# Autodesk Inventor assembly: TBone Cart
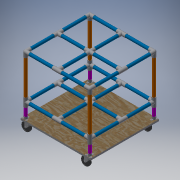
[picture p0: Inventor's stored thumbnail of the model, 180x180]
Saved by Autodesk Inventor 2018.2 (Build 222227000, 227)
## iProperties
Created: 2018-02-01
Part Number: TBone Cart
Document SubType Name: Assembly
Designer: owner
Author: owner
## Documents named in this file (11)
- Z:\The Pickle - 4 - Copy\Final Carts\T-Bone Cart\T-Bone Cart.iam
- Z:\The Pickle - 4 - Copy\Final Carts\Stuff Used By All Carts\PVC Fittings (Formufit)\4-way Tee 1 Inch.ipt
- Z:\The Pickle - 4 - Copy\Final Carts\Stuff Used By All Carts\PVC Fittings (Formufit)\Tee 1 Inch.ipt
- Z:\The Pickle - 4 - Copy\Final Carts\Stuff Used By All Carts\PVC Fittings (Formufit)\Cross 1 Inch.ipt
- Z:\The Pickle - 4 - Copy\Final Carts\Stuff Used By All Carts\PVC Fittings (Formufit)\Wood Mount 1 Inch.ipt
- Z:\The Pickle\Final Carts\T-Bone Cart\Pipe 1.ipt
- Z:\The Pickle\Final Carts\T-Bone Cart\Pipe 2.ipt
- Z:\The Pickle\Final Carts\T-Bone Cart\Pipe 3.ipt
- Z:\The Pickle - 4 - Copy\Final Carts\Stuff Used By All Carts\WHEELS.ipt
- Z:\The Pickle - 4 - Copy\Final Carts\Stuff Used By All Carts\PVC Fittings (Formufit)\3-way 90 1 Inch.ipt
- Z:\The Pickle - 4 - Copy\Final Carts\T-Bone Cart\T-Bone Plywood Base.ipt
## Components (59 placed, 10 different names)
1. T-Bone Plywood Base:1 — Mate:1, Tangent:1, Tangent:2, Flush:8, Flush:9, Flush:10, Flush:11, Mate:2, Tangent:3, Tangent:4, Tangent:5, Tangent:6, Tangent:7, Angle:1
2. 4-way Tee 1 Inch:1 — Insert:11, Insert:12, Insert:29, Insert:33
3. 4-way Tee 1 Inch:2 — Insert:7, Insert:8, Insert:28, Insert:32
4. 4-way Tee 1 Inch:3 — Insert:2, Insert:3, Insert:4, Insert:19
5. 4-way Tee 1 Inch:4 — Insert:15, Insert:16, Insert:30, Insert:31
6. Tee 1 Inch:1 — Insert:46, Insert:53
7. Tee 1 Inch:2 — Insert:13, Insert:14, Insert:21
8. Tee 1 Inch:3 — Insert:17, Insert:18, Insert:22
9. Tee 1 Inch:4 — Insert:47, Insert:52
10. Tee 1 Inch:5 — Insert:5, Insert:6, Insert:20
11. Tee 1 Inch:6 — Insert:49, Insert:51
12. Tee 1 Inch:7 — Insert:48, Insert:50
13. Tee 1 Inch:8 — Insert:9, Insert:10, Insert:23
14. Cross 1 Inch:1 — Insert:54, Insert:59
15. Cross 1 Inch:2 — Insert:24
16. Wood Mount 1 Inch:1 — Insert:25, Tangent:6
17. Wood Mount 1 Inch:2 — Insert:27, Tangent:4, Tangent:5
18. Wood Mount 1 Inch:3 — Insert:26, Tangent:7
19. Wood Mount 1 Inch:4 — Mate:1, Tangent:1, Tangent:2, Insert:1, Tangent:3
20. Pipe 1:1 — Insert:4, Insert:5
21. Pipe 1:2 — Insert:6, Insert:7
22. Pipe 1:3 — Insert:12, Insert:13
23. Pipe 1:4 — Insert:14, Insert:15
24. Pipe 1:5 — Insert:22, Insert:24
25. Pipe 1:6 — Insert:23
26. Pipe 1:7 — Insert:49, Tangent:8
27. Pipe 1:8
28. Pipe 1:9 — Insert:46
29. Pipe 1:10
30. Pipe 1:11 — Insert:50, Insert:54
31. Pipe 1:12 — Insert:52, Insert:59
32. Pipe 1:13 — Insert:8, Insert:9
33. Pipe 1:14 — Insert:10, Insert:11
34. Pipe 1:15 — Insert:16, Insert:17
35. Pipe 1:16 — Insert:18, Insert:19
36. Pipe 1:17 — Insert:20
37. Pipe 1:18
38. Pipe 1:19 — Insert:47
39. Pipe 1:20 — Insert:48
40. Pipe 1:21 — Insert:53
41. Pipe 1:22 — Insert:51
42. Pipe 1:23
43. Pipe 1:24 — Insert:21
44. Pipe 2:1 — Insert:1, Insert:2
45. Pipe 2:2 — Insert:27, Insert:30
46. Pipe 2:3 — Insert:26, Insert:29
47. Pipe 2:4 — Insert:25, Insert:28
48. Pipe 3:1 — Insert:3, Insert:58
49. Pipe 3:2 — Insert:31, Insert:55
50. Pipe 3:3 — Insert:32, Insert:57
51. Pipe 3:4 — Insert:33, Insert:56
52. WHEELS:1 — Flush:1, Flush:2, Flush:5, Flush:6, Flush:10
53. WHEELS:2 — Flush:2, Flush:3, Flush:6, Flush:7, Flush:11, Mate:2
54. WHEELS:3 — Flush:1, Flush:4, Flush:5, Flush:8, Flush:9
55. WHEELS:4 — Flush:3, Flush:4, Flush:7
56. 3-way 90 1 Inch:1 — Insert:56
57. 3-way 90 1 Inch:2 — Insert:57
58. 3-way 90 1 Inch:3 — Insert:58
59. 3-way 90 1 Inch:4 — Insert:55
## Relationships (69: Insert 47, Flush 11, Tangent 8, Mate 2, Angle 1)
- Mate:1: T-Bone Plywood Base:1 ↔ Wood Mount 1 Inch:4
- Tangent:1: T-Bone Plywood Base:1 ↔ Wood Mount 1 Inch:4
- Tangent:2: T-Bone Plywood Base:1 ↔ Wood Mount 1 Inch:4
- Insert:1: Wood Mount 1 Inch:4 ↔ Pipe 2:1
- Insert:2: 4-way Tee 1 Inch:3 ↔ Pipe 2:1
- Insert:3: 4-way Tee 1 Inch:3 ↔ Pipe 3:1
- Insert:4: 4-way Tee 1 Inch:3 ↔ Pipe 1:1
- Insert:5: Tee 1 Inch:5 ↔ Pipe 1:1
- Insert:6: Tee 1 Inch:5 ↔ Pipe 1:2
- Insert:7: 4-way Tee 1 Inch:2 ↔ Pipe 1:2
- Insert:8: 4-way Tee 1 Inch:2 ↔ Pipe 1:13
- Insert:9: Tee 1 Inch:8 ↔ Pipe 1:13
- Insert:10: Tee 1 Inch:8 ↔ Pipe 1:14
- Insert:11: 4-way Tee 1 Inch:1 ↔ Pipe 1:14
- Insert:12: 4-way Tee 1 Inch:1 ↔ Pipe 1:3
- Insert:13: Tee 1 Inch:2 ↔ Pipe 1:3
- Insert:14: Tee 1 Inch:2 ↔ Pipe 1:4
- Insert:15: 4-way Tee 1 Inch:4 ↔ Pipe 1:4
- Insert:16: 4-way Tee 1 Inch:4 ↔ Pipe 1:15
- Insert:17: Tee 1 Inch:3 ↔ Pipe 1:15
- Insert:18: Tee 1 Inch:3 ↔ Pipe 1:16
- Insert:19: 4-way Tee 1 Inch:3 ↔ Pipe 1:16
- Insert:20: Tee 1 Inch:5 ↔ Pipe 1:17
- Insert:21: Tee 1 Inch:2 ↔ Pipe 1:24
- Insert:22: Tee 1 Inch:3 ↔ Pipe 1:5
- Insert:23: Tee 1 Inch:8 ↔ Pipe 1:6
- Insert:24: Cross 1 Inch:2 ↔ Pipe 1:5
- Insert:25: Wood Mount 1 Inch:1 ↔ Pipe 2:4
- Insert:26: Wood Mount 1 Inch:3 ↔ Pipe 2:3
- Insert:27: Wood Mount 1 Inch:2 ↔ Pipe 2:2
- Insert:28: 4-way Tee 1 Inch:2 ↔ Pipe 2:4
- Insert:29: 4-way Tee 1 Inch:1 ↔ Pipe 2:3
- Insert:30: 4-way Tee 1 Inch:4 ↔ Pipe 2:2
- Insert:31: 4-way Tee 1 Inch:4 ↔ Pipe 3:2
- Insert:32: 4-way Tee 1 Inch:2 ↔ Pipe 3:3
- Insert:33: 4-way Tee 1 Inch:1 ↔ Pipe 3:4
- Insert:46: Tee 1 Inch:1 ↔ Pipe 1:9
- Insert:47: Tee 1 Inch:4 ↔ Pipe 1:19
- Insert:48: Tee 1 Inch:7 ↔ Pipe 1:20
- Insert:49: Tee 1 Inch:6 ↔ Pipe 1:7
- Insert:50: Tee 1 Inch:7 ↔ Pipe 1:11
- Insert:51: Tee 1 Inch:6 ↔ Pipe 1:22
- Insert:52: Tee 1 Inch:4 ↔ Pipe 1:12
- Insert:53: Tee 1 Inch:1 ↔ Pipe 1:21
- Insert:54: Cross 1 Inch:1 ↔ Pipe 1:11
- Flush:1: WHEELS:1 ↔ WHEELS:3
- Flush:2: WHEELS:1 ↔ WHEELS:2
- Flush:3: WHEELS:2 ↔ WHEELS:4
- Flush:4: WHEELS:3 ↔ WHEELS:4
- Flush:5: WHEELS:1 ↔ WHEELS:3
- Flush:6: WHEELS:1 ↔ WHEELS:2
- Flush:7: WHEELS:2 ↔ WHEELS:4
- Flush:8 (12.7 mm): T-Bone Plywood Base:1 ↔ WHEELS:3
- Flush:9 (12.7 mm): T-Bone Plywood Base:1 ↔ WHEELS:3
- Flush:10 (12.7 mm): T-Bone Plywood Base:1 ↔ WHEELS:1
- Flush:11 (12.7 mm): T-Bone Plywood Base:1 ↔ WHEELS:2
- Mate:2: T-Bone Plywood Base:1 ↔ WHEELS:2
- Insert:55: Pipe 3:2 ↔ 3-way 90 1 Inch:4
- Insert:56: Pipe 3:4 ↔ 3-way 90 1 Inch:1
- Insert:57: Pipe 3:3 ↔ 3-way 90 1 Inch:2
- Insert:58: Pipe 3:1 ↔ 3-way 90 1 Inch:3
- Tangent:3: T-Bone Plywood Base:1 ↔ Wood Mount 1 Inch:4
- Tangent:4: T-Bone Plywood Base:1 ↔ Wood Mount 1 Inch:2
- Tangent:5: T-Bone Plywood Base:1 ↔ Wood Mount 1 Inch:2
- Tangent:6: T-Bone Plywood Base:1 ↔ Wood Mount 1 Inch:1
- Tangent:7: T-Bone Plywood Base:1 ↔ Wood Mount 1 Inch:3
- Angle:1 (0 deg): T-Bone Plywood Base:1
- Tangent:8: Pipe 1:7
- Insert:59: Cross 1 Inch:1 ↔ Pipe 1:12
